# Autodesk Inventor assembly: 2924-1015-1000 assembly
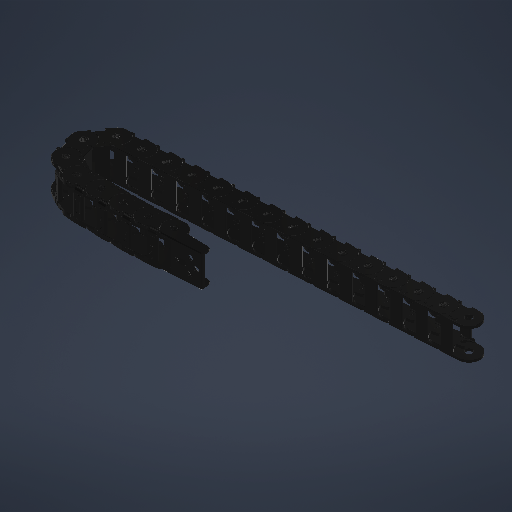
[picture p0: Inventor's stored thumbnail of the model, 512x512]
Saved by Autodesk Inventor 2026.2 (Build 302298000, 298)
## iProperties
Created: 2023-10-18
Part Number: 2924-1015-1000 assembly
Description: STEP AP203
Document SubType Name: Assembly
Designer: Kenji
Sending System: SolidWorks 2016
Preprocessor: SwSTEP 2.0
Title: 2924-1015-1000 assembly.STEP
Revision Number: ANY
## Documents named in this file (3)
- C:\Users\Kenji\Documents\GitHub\DiyCNC-\COTS-Parts\10x15-CableCarrierYAxis-2924-1015-1000.iam
- C:\Users\Kenji\Downloads\2924-1015-1000\2924-1015-1000 assembly\2924-1015-1000 assembly\2924-1015 link.ipt
- C:\Users\Kenji\Downloads\2924-1015-1000\2924-1015-1000 assembly\2924-1015-1000 assembly\2924-1015 End 2.ipt
## Components (22 placed, 16 different names)
1. 2924-1015 link_45 — Rotational:13, Rotational:14, Flush:8, Flush:9
2. 2924-1015 link_46 — Rotational:12, Rotational:13, Flush:7, Flush:8
3. 2924-1015 link_47 — Rotational:11, Rotational:12, Flush:6, Flush:7
4. 2924-1015 link_48 — Rotational:10, Rotational:11, Flush:5, Flush:6
5. 2924-1015 link_49 — Rotational:9, Rotational:10, Flush:4, Flush:5
6. 2924-1015 link_50 — Rotational:8, Rotational:9, Flush:4
7. 2924-1015 link_51 — Rotational:7, Rotational:8, Angle:4
8. 2924-1015 link_52 — Rotational:6, Rotational:7
9. 2924-1015 link_53 — Rotational:5, Rotational:6
10. 2924-1015 link_54 — Rotational:4, Rotational:5
11. 2924-1015 link_55 — Rotational:3, Rotational:4
12. 2924-1015 link_56 — Rotational:2, Rotational:3
13. 2924-1015 link_57 — Rotational:1, Rotational:2
14. 2924-1015 link_58 — Rotational:1, Mate:9, Mate:10
15. 2924-1015 End 2_59 — Mate:9, Mate:10, Angle:4
16. 2924-1015 link:58 — Rotational:14, Flush:9, Mate:3, Flush:10, Mate:6
17. 2924-1015 link:59 — Mate:3, Flush:10, Mate:4, Flush:11, Mate:6, Mate:7
18. 2924-1015 link:60 — Mate:4, Flush:11, Mate:5, Mate:7, Mate:8, Flush:12
19. 2924-1015 link:61 — Mate:5, Mate:8, Flush:12, Mate:11, Flush:13, Mate:12
20. 2924-1015 link:62 — Mate:11, Flush:13, Mate:12, Mate:13, Flush:14, Mate:14
21. 2924-1015 link:63 — Mate:13, Flush:14, Mate:14, Mate:15, Mate:16, Flush:15
22. 2924-1015 link:64 — Mate:15, Mate:16, Flush:15
## Relationships (41: RevoluteJoint 14, Mate 14, Flush 12, Angle 1)
- Rotational:1 [RevoluteJoint]: 2924-1015 link_57 ↔ 2924-1015 link_58
- Rotational:2 [RevoluteJoint]: 2924-1015 link_56 ↔ 2924-1015 link_57
- Rotational:3 [RevoluteJoint]: 2924-1015 link_55 ↔ 2924-1015 link_56
- Rotational:4 [RevoluteJoint]: 2924-1015 link_54 ↔ 2924-1015 link_55
- Rotational:5 [RevoluteJoint]: 2924-1015 link_53 ↔ 2924-1015 link_54
- Rotational:6 [RevoluteJoint]: 2924-1015 link_52 ↔ 2924-1015 link_53
- Rotational:7 [RevoluteJoint]: 2924-1015 link_51 ↔ 2924-1015 link_52
- Rotational:8 [RevoluteJoint]: 2924-1015 link_50 ↔ 2924-1015 link_51
- Rotational:9 [RevoluteJoint]: 2924-1015 link_49 ↔ 2924-1015 link_50
- Rotational:10 [RevoluteJoint]: 2924-1015 link_48 ↔ 2924-1015 link_49
- Rotational:11 [RevoluteJoint]: 2924-1015 link_47 ↔ 2924-1015 link_48
- Rotational:12 [RevoluteJoint]: 2924-1015 link_46 ↔ 2924-1015 link_47
- Rotational:13 [RevoluteJoint]: 2924-1015 link_45 ↔ 2924-1015 link_46
- Rotational:14 [RevoluteJoint]: 2924-1015 link_45 ↔ 2924-1015 link:58
- Flush:4: 2924-1015 link_49 ↔ 2924-1015 link_50
- Flush:5: 2924-1015 link_48 ↔ 2924-1015 link_49
- Flush:6: 2924-1015 link_47 ↔ 2924-1015 link_48
- Flush:7: 2924-1015 link_46 ↔ 2924-1015 link_47
- Flush:8: 2924-1015 link_45 ↔ 2924-1015 link_46
- Flush:9: 2924-1015 link_45 ↔ 2924-1015 link:58
- Mate:3: 2924-1015 link:58 ↔ 2924-1015 link:59
- Flush:10: 2924-1015 link:58 ↔ 2924-1015 link:59
- Mate:4: 2924-1015 link:59 ↔ 2924-1015 link:60
- Flush:11: 2924-1015 link:59 ↔ 2924-1015 link:60
- Mate:5: 2924-1015 link:60 ↔ 2924-1015 link:61
- Mate:6: 2924-1015 link:58 ↔ 2924-1015 link:59
- Mate:7: 2924-1015 link:59 ↔ 2924-1015 link:60
- Mate:8: 2924-1015 link:60 ↔ 2924-1015 link:61
- Flush:12: 2924-1015 link:60 ↔ 2924-1015 link:61
- Mate:9: 2924-1015 link_58 ↔ 2924-1015 End 2_59
- Mate:10: 2924-1015 link_58 ↔ 2924-1015 End 2_59
- Angle:4 (0 deg): 2924-1015 link_51 ↔ 2924-1015 End 2_59
- Mate:11: 2924-1015 link:61 ↔ 2924-1015 link:62
- Flush:13: 2924-1015 link:61 ↔ 2924-1015 link:62
- Mate:12: 2924-1015 link:61 ↔ 2924-1015 link:62
- Mate:13: 2924-1015 link:62 ↔ 2924-1015 link:63
- Flush:14: 2924-1015 link:62 ↔ 2924-1015 link:63
- Mate:14: 2924-1015 link:62 ↔ 2924-1015 link:63
- Mate:15: 2924-1015 link:63 ↔ 2924-1015 link:64
- Mate:16: 2924-1015 link:63 ↔ 2924-1015 link:64
- Flush:15: 2924-1015 link:63 ↔ 2924-1015 link:64
